# Autodesk Inventor assembly: BATTERY ASSEMBLY
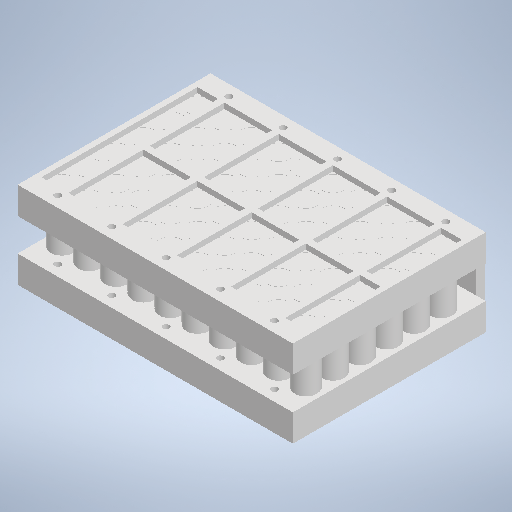
[picture p0: Inventor's stored thumbnail of the model, 512x512]
Saved by Autodesk Inventor 2025.2 (Build 292293000, 293)
## iProperties
Created: 2025-03-22
Part Number: BATTERY ASSEMBLY
Document SubType Name: Assembly
Designer: Mathias
Author: Mathias
## Documents named in this file (5)
- C:\Users\Mathias B. Kampp\Desktop\Uni\Project_ØK\Inventor\Autodesk-inventor-filesharing\BATTERY ASSEMBLY.iam
- C:\Users\Mathias B. Kampp\Desktop\Uni\Project_ØK\Inventor\Autodesk-inventor-filesharing\21700.ipt
- C:\Users\Mathias B. Kampp\Desktop\Uni\Project_ØK\Inventor\Autodesk-inventor-filesharing\BMS.ipt
- C:\Users\Mathias B. Kampp\Desktop\Uni\Project_ØK\Inventor\Autodesk-inventor-filesharing\Battery Holder pt1.ipt
- C:\Users\Mathias B. Kampp\Desktop\Uni\Project_ØK\Inventor\Autodesk-inventor-filesharing\Battery Holder pt2.ipt
## Components (63 placed, 4 different names)
1. BMS:1 — Mate:1
2. Battery Holder pt1:1 — Insert:1, Mate:1
3. Battery Holder pt2:1 — Insert:2
4. 21700:1
5. 21700:2
6. 21700:3
7. 21700:4
8. 21700:5
9. 21700:6
10. 21700:7
11. 21700:8
12. 21700:9
13. 21700:10
14. 21700:11
15. 21700:12
16. 21700:13
17. 21700:14
18. 21700:15
19. 21700:16
20. 21700:17
21. 21700:18
22. 21700:19
23. 21700:20
24. 21700:21
25. 21700:22
26. 21700:23
27. 21700:24
28. 21700:25
29. 21700:26
30. 21700:27
31. 21700:28
32. 21700:29
33. 21700:30
34. 21700:31
35. 21700:32
36. 21700:33
37. 21700:34
38. 21700:35
39. 21700:36
40. 21700:37
41. 21700:38
42. 21700:39
43. 21700:40
44. 21700:41
45. 21700:42
46. 21700:43
47. 21700:44
48. 21700:45
49. 21700:46
50. 21700:47
51. 21700:48
52. 21700:49
53. 21700:50
54. 21700:51 — Insert:1
55. 21700:52 — Insert:2
56. 21700:53
57. 21700:54
58. 21700:55
59. 21700:56
60. 21700:57
61. 21700:58
62. 21700:59
63. 21700:60
## Component patterns: (60 elements, first: 21700:1)
## Relationships (3: Insert 2, Mate 1)
- Insert:1: Battery Holder pt1:1 ↔ 21700:51
- Insert:2: Battery Holder pt2:1 ↔ 21700:52
- Mate:1: BMS:1 ↔ Battery Holder pt1:1
